# Autodesk Inventor assembly: 上下直動
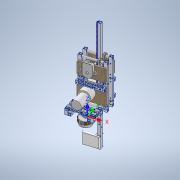
[picture p0: Inventor's stored thumbnail of the model, 180x180]
Saved by Autodesk Inventor 2020.3 (Build 243373000, 373)
## iProperties
Created: 2020-07-05
Part Number: 上下直動
Document SubType Name: Assembly
Designer: totot
Mass: 467.946 g
Surface Area: 1548.91 cm^2
Volume: 213.509 cm^3
Density: 2.19169 g/cm^3
Author: totot
## Documents named in this file (24)
- D:\mysvn\ロボコン\キャチロボ\キャチロボ設計図\ロボット\上下直動\上下直動.iam
- D:\mysvn\ロボコン\キャチロボ\キャチロボ設計図\ロボット\ハンド\フランジ.ipt
- D:\mysvn\ロボコン\キャチロボ\キャチロボ設計図\ロボット\上下直動\上下直動9x9_1.ipt
- D:\mysvn\ロボコン\キャチロボ\キャチロボ設計図\ロボット\上下直動\上下直動9x9_2.ipt
- D:\mysvn\ロボコン\キャチロボ\キャチロボ設計図\ロボット\上下直動\上下直動9x9_3.ipt
- D:\mysvn\ロボコン\キャチロボ\キャチロボ設計図\ロボット\上下直動\上下直動9x9x18.ipt
- D:\mysvn\ロボコン\キャチロボ\キャチロボ設計図\ロボット\上下直動\上下直動9x9_1_CPY.ipt
- D:\mysvn\ロボコン\キャチロボ\キャチロボ設計図\ロボット\上下直動\上下直動t5.5.ipt
- D:\mysvn\ロボコン\キャチロボ\キャチロボ設計図\ロボット\共有パーツ\PS1-20_On.ipt
- D:\mysvn\ロボコン\キャチロボ\キャチロボ設計図\ロボット\上下直動\上下直動_ベアリングシャフト.ipt
- D:\mysvn\ロボコン\キャチロボ\キャチロボ設計図\ロボット\共有パーツ\ベアリング_4-8.ipt
- D:\mysvn\ロボコン\キャチロボ\キャチロボ設計図\ロボット\上下直動\上下直動_ベアリングシャフト2.ipt
- D:\mysvn\ロボコン\キャチロボ\キャチロボ設計図\ロボット\共有パーツ\ベアリング_6-17.ipt
- D:\mysvn\ロボコン\キャチロボ\キャチロボ設計図\ロボット\上下直動\上下直動9x9_4.ipt
- D:\mysvn\ロボコン\キャチロボ\キャチロボ設計図\ロボット\上下直動\上下直動t5.5_エンコーダ軸受け.ipt
- D:\mysvn\ロボコン\キャチロボ\キャチロボ設計図\ロボット\共有パーツ\F606ZZ\F606ZZ.iam
- D:\mysvn\ロボコン\キャチロボ\キャチロボ設計図\ロボット\共有パーツ\AMT102-Vwide.ipt
- D:\mysvn\ロボコン\キャチロボ\キャチロボ設計図\ロボット\上下直動\上下直動t5.5_エンコーダ軸受け_CPY.ipt
- D:\mysvn\ロボコン\キャチロボ\キャチロボ設計図\ロボット\上下直動\上下直動_エンコーダシャフト.ipt
- D:\mysvn\ロボコン\キャチロボ\キャチロボ設計図\ロボット\共有パーツ\PS1-40_On.ipt
- D:\mysvn\ロボコン\キャチロボ\キャチロボ設計図\ロボット\共有パーツ\RS_380.ipt
- D:\mysvn\ロボコン\キャチロボ\キャチロボ設計図\ロボット\ハンド\ハンド9x9_4_CPY.ipt
- D:\mysvn\ロボコン\キャチロボ\キャチロボ設計図\ロボット\共有パーツ\DR1-2000_On3.ipt
- D:\mysvn\ロボコン\キャチロボ\キャチロボ設計図\ロボット\共有パーツ\ハンド3D_L_CPY.ipt
## Components (43 placed, 23 different names)
1. フランジ:1 — 挿入:1, 挿入:2, 挿入:3, 挿入:4, 正接:18, フラッシュ:12
2. 上下直動9x9_1:1 — 挿入:1, 挿入:2, 挿入:6, 挿入:8, 挿入:59, 挿入:61
3. 上下直動9x9_1:2 — 挿入:3, 挿入:4, 挿入:5, 挿入:7, 挿入:18, 挿入:23
4. 上下直動9x9_2:1 — 挿入:5, 挿入:6, 挿入:16, 挿入:17, 挿入:19, 挿入:25, 挿入:27, 挿入:60
5. 上下直動9x9_2:2 — 挿入:7, 挿入:8, 挿入:21, 挿入:22, 挿入:24, 挿入:28, 挿入:58
6. 上下直動9x9_3:1 — 挿入:21, 挿入:45, 挿入:54, 正接:12, 挿入:66
7. 上下直動9x9_3:2 — 挿入:16, 挿入:50, 挿入:57, 挿入:67, 挿入:70, 挿入:72
8. 上下直動9x9x18:1 — 挿入:22, 挿入:23
9. 上下直動9x9x18:2 — 挿入:17, 挿入:18
10. 上下直動9x9_3:3 — 挿入:19, フラッシュ:5, 挿入:40, 挿入:42, 挿入:56, 挿入:63, 挿入:71, フラッシュ:16
11. 上下直動9x9_3:4 — 挿入:24, メイト:2, 挿入:41, 挿入:53, フラッシュ:7, 正接:11, 挿入:62, メイト:5
12. 上下直動9x9_1_CPY:1 — 挿入:25, 挿入:27, 挿入:28, 挿入:42
13. 上下直動9x9_1_CPY:2 — 挿入:40, 挿入:41, 挿入:52, 挿入:55
14. 上下直動9x9_1_CPY:3 — 挿入:47, 挿入:48, 挿入:49, 挿入:51
15. 上下直動t5.5:1 — 挿入:38, 挿入:39, 挿入:45, 挿入:47, 挿入:48, 挿入:49, 挿入:50, 挿入:68, 挿入:69
16. PS1-20_On:1 — フラッシュ:1, フラッシュ:11, 正接:23
17. 上下直動_ベアリングシャフト:1 — 挿入:38, 正接:4
18. 上下直動_ベアリングシャフト:2 — 挿入:39, 正接:3
19. ベアリング_4-8:1 — 正接:3, フラッシュ:2
20. ベアリング_4-8:2 — 正接:4, フラッシュ:1, フラッシュ:2, 正接:26
21. 上下直動_ベアリングシャフト2:1 — 正接:8, 挿入:71
22. 上下直動_ベアリングシャフト2:2 — フラッシュ:5, 正接:7, 挿入:70
23. 上下直動_ベアリングシャフト2:3 — 正接:12, 正接:14, 挿入:72
24. 上下直動_ベアリングシャフト2:5 — フラッシュ:7, 正接:11, 正接:13
25. ベアリング_6-17:1 — 正接:8, フラッシュ:6, 正接:24
26. ベアリング_6-17:2 — 正接:7, メイト:2, フラッシュ:6, フラッシュ:9, 正接:25
27. 上下直動9x9_4:1 — 挿入:51, 挿入:52, 挿入:53, 挿入:54
28. 上下直動9x9_4:2 — 挿入:55, 挿入:56, 挿入:57
29. ベアリング_6-17:3 — フラッシュ:8, フラッシュ:9, 正接:14
30. ベアリング_6-17:4 — フラッシュ:8, 正接:13
31. 上下直動9x9x18:3 — 挿入:58, 挿入:59
32. 上下直動9x9x18:4 — 挿入:60, 挿入:61
33. 上下直動t5.5_エンコーダ軸受け:1 — 挿入:62, 挿入:63, 正接:15, メイト:3
34. F606ZZ:1 [sub-assembly] — 正接:15, メイト:3, フラッシュ:10, 正接:16
35. AMT102-Vwide:1 — 挿入:64, 挿入:65
36. 上下直動t5.5_エンコーダ軸受け_CPY:1 — 挿入:64, 挿入:65, 挿入:66, 挿入:67
37. 上下直動_エンコーダシャフト:1 — フラッシュ:10, 正接:16, 正接:17
38. PS1-20_On:2 — フラッシュ:11, 正接:17, フラッシュ:13
39. PS1-40_On:1 — 正接:18, フラッシュ:12
40. RS_380:1 — 挿入:68, 挿入:69, 正接:23, フラッシュ:13
41. ハンド9x9_4_CPY:1 — フラッシュ:14, メイト:4, フラッシュ:15, フラッシュ:16, メイト:5, 正接:24, 正接:25, 正接:26, 挿入:73, 挿入:74
42. DR1-2000_On3:1 — フラッシュ:14, メイト:4, フラッシュ:15
43. ハンド3D_L_CPY:1 — 挿入:73, 挿入:74
## Relationships (87: Insert 53, Tangent 16, Flush 14, Mate 4)
- 挿入:1 [Insert]: フランジ:1 ↔ 上下直動9x9_1:1
- 挿入:2 [Insert]: フランジ:1 ↔ 上下直動9x9_1:1
- 挿入:3 [Insert]: フランジ:1 ↔ 上下直動9x9_1:2
- 挿入:4 [Insert]: フランジ:1 ↔ 上下直動9x9_1:2
- 挿入:5 [Insert]: 上下直動9x9_1:2 ↔ 上下直動9x9_2:1
- 挿入:6 [Insert]: 上下直動9x9_1:1 ↔ 上下直動9x9_2:1
- 挿入:7 [Insert]: 上下直動9x9_1:2 ↔ 上下直動9x9_2:2
- 挿入:8 [Insert]: 上下直動9x9_1:1 ↔ 上下直動9x9_2:2
- 挿入:16 [Insert]: 上下直動9x9_2:1 ↔ 上下直動9x9_3:2
- 挿入:17 [Insert]: 上下直動9x9_2:1 ↔ 上下直動9x9x18:2
- 挿入:18 [Insert]: 上下直動9x9_1:2 ↔ 上下直動9x9x18:2
- 挿入:19 [Insert]: 上下直動9x9_2:1 ↔ 上下直動9x9_3:3
- 挿入:21 [Insert]: 上下直動9x9_2:2 ↔ 上下直動9x9_3:1
- 挿入:22 [Insert]: 上下直動9x9_2:2 ↔ 上下直動9x9x18:1
- 挿入:23 [Insert]: 上下直動9x9_1:2 ↔ 上下直動9x9x18:1
- 挿入:24 [Insert]: 上下直動9x9_2:2 ↔ 上下直動9x9_3:4
- 挿入:25 [Insert]: 上下直動9x9_2:1 ↔ 上下直動9x9_1_CPY:1
- 挿入:27 [Insert]: 上下直動9x9_2:1 ↔ 上下直動9x9_1_CPY:1
- 挿入:28 [Insert]: 上下直動9x9_2:2 ↔ 上下直動9x9_1_CPY:1
- 挿入:38 [Insert]: 上下直動t5.5:1 ↔ 上下直動_ベアリングシャフト:1
- 挿入:39 [Insert]: 上下直動t5.5:1 ↔ 上下直動_ベアリングシャフト:2
- 正接:3 [Tangent]: 上下直動_ベアリングシャフト:2 ↔ ベアリング_4-8:1
- 正接:4 [Tangent]: 上下直動_ベアリングシャフト:1 ↔ ベアリング_4-8:2
- フラッシュ:1 [Flush] (5 mm): PS1-20_On:1 ↔ ベアリング_4-8:2
- フラッシュ:2 [Flush]: ベアリング_4-8:1 ↔ ベアリング_4-8:2
- フラッシュ:5 [Flush]: 上下直動9x9_3:3 ↔ 上下直動_ベアリングシャフト2:2
- 正接:7 [Tangent]: 上下直動_ベアリングシャフト2:2 ↔ ベアリング_6-17:2
- 正接:8 [Tangent]: 上下直動_ベアリングシャフト2:1 ↔ ベアリング_6-17:1
- メイト:2 [Mate] (10 mm): 上下直動9x9_3:4 ↔ ベアリング_6-17:2
- フラッシュ:6 [Flush]: ベアリング_6-17:1 ↔ ベアリング_6-17:2
- 挿入:40 [Insert]: 上下直動9x9_3:3 ↔ 上下直動9x9_1_CPY:2
- 挿入:41 [Insert]: 上下直動9x9_3:4 ↔ 上下直動9x9_1_CPY:2
- 挿入:42 [Insert]: 上下直動9x9_3:3 ↔ 上下直動9x9_1_CPY:1
- 挿入:45 [Insert]: 上下直動9x9_3:1 ↔ 上下直動t5.5:1
- 挿入:47 [Insert]: 上下直動9x9_1_CPY:3 ↔ 上下直動t5.5:1
- 挿入:48 [Insert]: 上下直動9x9_1_CPY:3 ↔ 上下直動t5.5:1
- 挿入:49 [Insert]: 上下直動9x9_1_CPY:3 ↔ 上下直動t5.5:1
- 挿入:50 [Insert]: 上下直動9x9_3:2 ↔ 上下直動t5.5:1
- 挿入:51 [Insert]: 上下直動9x9_1_CPY:3 ↔ 上下直動9x9_4:1
- 挿入:52 [Insert]: 上下直動9x9_1_CPY:2 ↔ 上下直動9x9_4:1
- 挿入:53 [Insert]: 上下直動9x9_3:4 ↔ 上下直動9x9_4:1
- 挿入:54 [Insert]: 上下直動9x9_3:1 ↔ 上下直動9x9_4:1
- 挿入:55 [Insert]: 上下直動9x9_1_CPY:2 ↔ 上下直動9x9_4:2
- 挿入:56 [Insert]: 上下直動9x9_3:3 ↔ 上下直動9x9_4:2
- 挿入:57 [Insert]: 上下直動9x9_3:2 ↔ 上下直動9x9_4:2
- フラッシュ:7 [Flush]: 上下直動9x9_3:4 ↔ 上下直動_ベアリングシャフト2:5
- 正接:11 [Tangent]: 上下直動9x9_3:4 ↔ 上下直動_ベアリングシャフト2:5
- 正接:12 [Tangent]: 上下直動9x9_3:1 ↔ 上下直動_ベアリングシャフト2:3
- フラッシュ:8 [Flush]: ベアリング_6-17:3 ↔ ベアリング_6-17:4
- フラッシュ:9 [Flush]: ベアリング_6-17:2 ↔ ベアリング_6-17:3
- 正接:13 [Tangent]: 上下直動_ベアリングシャフト2:5 ↔ ベアリング_6-17:4
- 正接:14 [Tangent]: 上下直動_ベアリングシャフト2:3 ↔ ベアリング_6-17:3
- 挿入:58 [Insert]: 上下直動9x9_2:2 ↔ 上下直動9x9x18:3
- 挿入:59 [Insert]: 上下直動9x9_1:1 ↔ 上下直動9x9x18:3
- 挿入:60 [Insert]: 上下直動9x9_2:1 ↔ 上下直動9x9x18:4
- 挿入:61 [Insert]: 上下直動9x9_1:1 ↔ 上下直動9x9x18:4
- 挿入:62 [Insert]: 上下直動9x9_3:4 ↔ 上下直動t5.5_エンコーダ軸受け:1
- 挿入:63 [Insert]: 上下直動9x9_3:3 ↔ 上下直動t5.5_エンコーダ軸受け:1
- 挿入:64 [Insert]: AMT102-Vwide:1 ↔ 上下直動t5.5_エンコーダ軸受け_CPY:1
- 挿入:65 [Insert]: AMT102-Vwide:1 ↔ 上下直動t5.5_エンコーダ軸受け_CPY:1
- 挿入:66 [Insert]: 上下直動9x9_3:1 ↔ 上下直動t5.5_エンコーダ軸受け_CPY:1
- 挿入:67 [Insert]: 上下直動9x9_3:2 ↔ 上下直動t5.5_エンコーダ軸受け_CPY:1
- 正接:15 [Tangent]: 上下直動t5.5_エンコーダ軸受け:1 ↔ F606ZZ:1
- メイト:3 [Mate]: 上下直動t5.5_エンコーダ軸受け:1 ↔ F606ZZ:1
- フラッシュ:10 [Flush]: F606ZZ:1 ↔ 上下直動_エンコーダシャフト:1
- 正接:16 [Tangent]: F606ZZ:1 ↔ 上下直動_エンコーダシャフト:1
- フラッシュ:11 [Flush]: PS1-20_On:1 ↔ PS1-20_On:2
- 正接:17 [Tangent]: 上下直動_エンコーダシャフト:1 ↔ PS1-20_On:2
- 正接:18 [Tangent]: フランジ:1 ↔ PS1-40_On:1
- フラッシュ:12 [Flush]: フランジ:1 ↔ PS1-40_On:1
- 挿入:68 [Insert]: 上下直動t5.5:1 ↔ RS_380:1
- 挿入:69 [Insert]: 上下直動t5.5:1 ↔ RS_380:1
- 正接:23 [Tangent]: PS1-20_On:1 ↔ RS_380:1
- フラッシュ:13 [Flush] (3 mm): PS1-20_On:2 ↔ RS_380:1
- 挿入:70 [Insert]: 上下直動9x9_3:2 ↔ 上下直動_ベアリングシャフト2:2
- 挿入:71 [Insert]: 上下直動9x9_3:3 ↔ 上下直動_ベアリングシャフト2:1
- フラッシュ:14 [Flush] (1 mm): ハンド9x9_4_CPY:1 ↔ DR1-2000_On3:1
- メイト:4 [Mate]: ハンド9x9_4_CPY:1 ↔ DR1-2000_On3:1
- フラッシュ:15 [Flush]: ハンド9x9_4_CPY:1 ↔ DR1-2000_On3:1
- 挿入:72 [Insert]: 上下直動9x9_3:2 ↔ 上下直動_ベアリングシャフト2:3
- フラッシュ:16 [Flush]: 上下直動9x9_3:3 ↔ ハンド9x9_4_CPY:1
- メイト:5 [Mate] (4 mm): 上下直動9x9_3:4 ↔ ハンド9x9_4_CPY:1
- 正接:24 [Tangent]: ベアリング_6-17:1 ↔ ハンド9x9_4_CPY:1
- 正接:25 [Tangent]: ベアリング_6-17:2 ↔ ハンド9x9_4_CPY:1
- 正接:26 [Tangent]: ベアリング_4-8:2 ↔ ハンド9x9_4_CPY:1
- 挿入:73 [Insert]: ハンド9x9_4_CPY:1 ↔ ハンド3D_L_CPY:1
- 挿入:74 [Insert]: ハンド9x9_4_CPY:1 ↔ ハンド3D_L_CPY:1
